# Autodesk Inventor assembly: Shoulder Joint Assembly
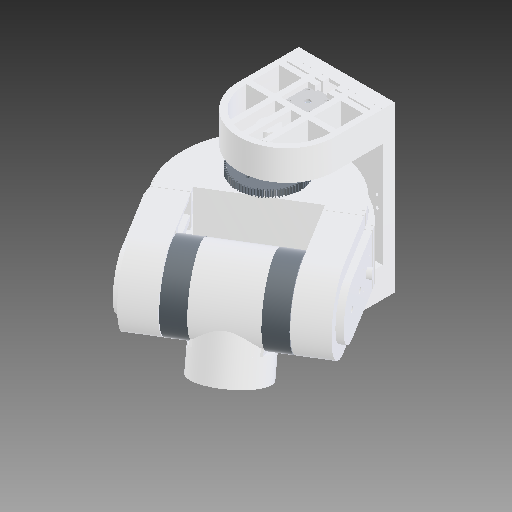
[picture p0: Inventor's stored thumbnail of the model, 512x512]
Saved by Autodesk Inventor 2017 SP1 (Build 210196100, 196)
## iProperties
Created: 2017-06-01
Part Number: Shoulder Joint Assembly
Document SubType Name: Assembly
Designer: Zach
Author: Zach
## Documents named in this file (22)
- C:\Users\Zach\Documents\GitHub\cr-laundry-robot\src\Body\Arm Assembly\Shoulder Joint Assembly\Shoulder Joint Assembly.iam
- C:\Users\Zach\Documents\GitHub\cr-laundry-robot\src\Body\Arm Assembly\Shoulder Joint Assembly\SJ002.ipt
- C:\Users\Zach\Documents\GitHub\cr-laundry-robot\src\Body\Arm Assembly\Shoulder Joint Assembly\SJ003.ipt
- C:\Users\Zach\Documents\GitHub\cr-laundry-robot\src\Body\Arm Assembly\Shoulder Joint Assembly\SJ001.ipt
- C:\Users\Zach\Documents\GitHub\cr-laundry-robot\lib\Stepper Motor - NEMA 17\NEMA17.ipt
- C:\Users\Zach\Documents\GitHub\cr-laundry-robot\src\Body\Arm Assembly\Shoulder Joint Assembly\SJ004.ipt
- C:\Users\Zach\Documents\GitHub\cr-laundry-robot\src\Body\Arm Assembly\Shoulder Joint Assembly\SJ005.ipt
- C:\Users\Zach\Documents\GitHub\cr-laundry-robot\src\Body\Arm Assembly\Shoulder Joint Assembly\SJ006.ipt
- C:\Users\Zach\Documents\GitHub\cr-laundry-robot\lib\U51105\U51105.ipt
- C:\Users\Zach\Documents\GitHub\cr-laundry-robot\lib\QS12MM250\QS12MM250.ipt
- C:\Users\Zach\Documents\GitHub\cr-laundry-robot\lib\6201RS\6201RS.ipt
- C:\Users\Zach\Documents\GitHub\cr-laundry-robot\src\Body\Arm Assembly\Shoulder Joint Assembly\SJ007.ipt
- C:\Users\Zach\Documents\GitHub\cr-laundry-robot\src\Body\Arm Assembly\Shoulder Joint Assembly\SJ008.ipt
- C:\Users\Zach\Documents\GitHub\cr-laundry-robot\src\Body\Arm Assembly\Shoulder Joint Assembly\Shoulder Joint Assembly\Design Accelerator\Spur Gears1.iam
- C:\Users\Zach\Documents\GitHub\cr-laundry-robot\src\Body\Arm Assembly\Shoulder Joint Assembly\SJ009.ipt
- C:\Users\Zach\Documents\GitHub\cr-laundry-robot\lib\Strain Wave Gearbox\StrainWaveGearbox.iam
- C:\Users\Zach\Documents\GitHub\cr-laundry-robot\src\Body\Arm Assembly\Shoulder Joint Assembly\Motor Gear.ipt
- C:\Users\Zach\Documents\GitHub\cr-laundry-robot\src\Body\Arm Assembly\Shoulder Joint Assembly\Motor Coupler.ipt
- C:\Users\Zach\Documents\GitHub\cr-laundry-robot\src\Body\Arm Assembly\Shoulder Joint Assembly\SJ013.ipt
- C:\Users\Zach\Documents\GitHub\cr-laundry-robot\src\Body\Arm Assembly\Shoulder Joint Assembly\SJ014.ipt
- C:\Users\Zach\Documents\GitHub\cr-laundry-robot\src\Body\Arm Assembly\Shoulder Joint Assembly\SJ016.ipt
- C:\Users\Zach\Documents\GitHub\cr-laundry-robot\lib\22x8x8mm Bearing.ipt
## Components (41 placed, 21 different names)
1. SJ001:1 — Mate:47, Mate:173, Mate:176, Mate:223, Mate:227, Mate:228, Mate:229, Mate:230, Mate:231, Mate:232, Mate:234, Mate:235
2. SJ001:2 — Mate:162, Mate:168, Mate:169, Mate:170, Mate:199, Mate:201, Mate:202, Mate:204, Mate:205, Mate:206, Mate:208, Mate:209, Mate:210, Mate:211, Mate:219
3. SJ002:1 — Mate:1, Mate:4, Mate:8, Mate:9, Mate:174, Mate:178
4. SJ002:2 — Mate:18, Mate:19, Mate:20, Mate:172
5. SJ003:1 — Mate:1, Mate:4, Mate:8, Mate:9, Mate:18, Mate:19, Mate:20, Mate:148, Mate:149, Mate:150, Mate:164, Mate:165, Mate:166, Mate:167, Mate:179, Mate:180, Mate:182
6. SJ004:1 — Mate:130, Mate:162, Mate:163, Mate:209, Mate:210, Mate:211, Mate:212, Mate:213, Mate:214
7. SJ004:2 — Mate:47, Mate:54, Mate:55, Mate:56, Mate:216, Mate:217
8. SJ005:1 — Mate:54, Mate:55, Mate:56, Mate:60, Mate:67, Mate:69, Mate:70, Mate:80, Flush:1, Mate:218
9. SJ005:2 — Mate:68, Mate:82, Mate:84, Mate:130, Mate:136, Flush:1, Mate:163, Mate:214, Mate:218
10. SJ006:2 — Mate:67, Mate:68, Mate:69, Mate:70, Mate:78, Mate:79, Mate:83
11. NEMA17:3 — Mate:148, Mate:149, Mate:150, Mate:181
12. U51105:1 — Mate:131, Mate:139, Mate:215
13. U51105:2 — Mate:78, Mate:79
14. QS12MM250:1 — Mate:80, Mate:105, Mate:117, Mate:119, Mate:120, Mate:132, Mate:134, Mate:215
15. 6201RS:1 — Mate:82, Mate:138
16. 6201RS:2 — Mate:83, Mate:84
17. SJ007:1 — Mate:121, Mate:122, Mate:123, Mate:133
18. SJ008:1 — Mate:119, Mate:125, Mate:126, Mate:127, Mate:132
19. SJ008:2 — Mate:97, Mate:98, Mate:99, Mate:105, Mate:112, Mate:117, Mate:120, Mate:121, Mate:122, Mate:123, Mate:124, Mate:131
20. NEMA17:4 — Mate:97, Mate:98, Mate:99, Mate:137
21. SJ007:2 — Mate:125, Mate:126, Mate:127, Mate:133
22. Spur Gears:1 [sub-assembly] — Mate:134, Mate:136, Mate:137, Mate:138, Mate:139
23. SJ009:1 — Mate:212, Mate:213
24. SJ009:2 — Mate:216, Mate:217
25. StrainWaveGearbox:1 [sub-assembly] — Mate:164, Mate:165, Mate:166
26. StrainWaveGearbox:2 [sub-assembly] — Mate:167, Mate:168, Mate:169, Mate:170, Mate:172
27. StrainWaveGearbox:3 [sub-assembly] — Mate:173, Mate:174, Mate:176, Mate:178
28. Motor Gear:1 — Mate:181, Mate:182, Rotation:1
29. Motor Coupler:1 — Mate:179, Mate:180, Rotation:1
30. SJ013:1 — Mate:203, Mate:204, Mate:207
31. SJ014:1 — Mate:202, Mate:219, Mate:220, Mate:221
32. NEMA17:5 — Mate:199, Mate:201, Mate:203, Mate:207, Mate:208
33. SJ016:1 — Mate:205, Mate:206, Mate:222, Flush:2
34. 22x8x8mm Bearing:1 — Mate:222, Flush:2
35. 22x8x8mm Bearing:2 — Mate:220, Mate:221
36. SJ013:2 — Mate:229, Mate:230
37. SJ014:2 — Mate:223, Mate:224, Mate:225, Mate:231
38. SJ016:2 — Mate:226, Flush:3, Mate:227, Mate:228
39. 22x8x8mm Bearing:4 — Mate:226, Flush:3
40. 22x8x8mm Bearing:5 — Mate:224, Mate:225
41. NEMA17:6 — Mate:232, Mate:234, Mate:235
## Relationships (106: Mate 102, Flush 3, RelateRotation 1)
- Mate:1: SJ002:1 ↔ SJ003:1
- Mate:4: SJ002:1 ↔ SJ003:1
- Mate:8: SJ002:1 ↔ SJ003:1
- Mate:9: SJ002:1 ↔ SJ003:1
- Mate:18: SJ002:2 ↔ SJ003:1
- Mate:19: SJ002:2 ↔ SJ003:1
- Mate:20: SJ002:2 ↔ SJ003:1
- Mate:47: SJ001:1 ↔ SJ004:2
- Mate:54: SJ004:2 ↔ SJ005:1
- Mate:55: SJ004:2 ↔ SJ005:1
- Mate:56: SJ004:2 ↔ SJ005:1
- Mate:60: SJ005:1
- Mate:67: SJ005:1 ↔ SJ006:2
- Mate:68: SJ005:2 ↔ SJ006:2
- Mate:69: SJ005:1 ↔ SJ006:2
- Mate:70: SJ005:1 ↔ SJ006:2
- Mate:78: SJ006:2 ↔ U51105:2
- Mate:79: SJ006:2 ↔ U51105:2
- Mate:80: SJ005:1 ↔ QS12MM250:1
- Mate:82: SJ005:2 ↔ 6201RS:1
- Mate:83: SJ006:2 ↔ 6201RS:2
- Mate:84: SJ005:2 ↔ 6201RS:2
- Mate:97: SJ008:2 ↔ NEMA17:4
- Mate:98: SJ008:2 ↔ NEMA17:4
- Mate:99: SJ008:2 ↔ NEMA17:4
- Mate:105: QS12MM250:1 ↔ SJ008:2
- Mate:112: SJ008:2
- Mate:117: QS12MM250:1 ↔ SJ008:2
- Mate:119: QS12MM250:1 ↔ SJ008:1
- Mate:120: QS12MM250:1 ↔ SJ008:2
- Mate:121: SJ007:1 ↔ SJ008:2
- Mate:122: SJ007:1 ↔ SJ008:2
- Mate:123: SJ007:1 ↔ SJ008:2
- Mate:124: SJ008:2
- Mate:125: SJ008:1 ↔ SJ007:2
- Mate:126: SJ008:1 ↔ SJ007:2
- Mate:127: SJ008:1 ↔ SJ007:2
- Mate:130: SJ004:1 ↔ SJ005:2
- Mate:131: U51105:1 ↔ SJ008:2
- Mate:132: QS12MM250:1 ↔ SJ008:1
- Mate:133: SJ007:1 ↔ SJ007:2
- Mate:134: QS12MM250:1 ↔ Spur Gears:1
- Mate:136: SJ005:2 ↔ Spur Gears:1
- Mate:137: NEMA17:4 ↔ Spur Gears:1
- Mate:138: 6201RS:1 ↔ Spur Gears:1
- Mate:139: U51105:1 ↔ Spur Gears:1
- Mate:148: SJ003:1 ↔ NEMA17:3
- Mate:149: SJ003:1 ↔ NEMA17:3
- Mate:150: SJ003:1 ↔ NEMA17:3
- Mate:162: SJ001:2 ↔ SJ004:1
- Flush:1: SJ005:1 ↔ SJ005:2
- Mate:163: SJ004:1 ↔ SJ005:2
- Mate:164: SJ003:1 ↔ StrainWaveGearbox:1
- Mate:165: SJ003:1 ↔ StrainWaveGearbox:1
- Mate:166: SJ003:1 ↔ StrainWaveGearbox:1
- Mate:167: SJ003:1 ↔ StrainWaveGearbox:2
- Mate:168: SJ001:2 ↔ StrainWaveGearbox:2
- Mate:169: SJ001:2 ↔ StrainWaveGearbox:2
- Mate:170: SJ001:2 ↔ StrainWaveGearbox:2
- Mate:172: SJ002:2 ↔ StrainWaveGearbox:2
- Mate:173: SJ001:1 ↔ StrainWaveGearbox:3
- Mate:174: SJ002:1 ↔ StrainWaveGearbox:3
- Mate:176: SJ001:1 ↔ StrainWaveGearbox:3
- Mate:178: SJ002:1 ↔ StrainWaveGearbox:3
- Mate:179: SJ003:1 ↔ Motor Coupler:1
- Mate:180: SJ003:1 ↔ Motor Coupler:1
- Mate:181: NEMA17:3 ↔ Motor Gear:1
- Mate:182: SJ003:1 ↔ Motor Gear:1
- Rotation:1 [RelateRotation] (1 ul): Motor Gear:1 ↔ Motor Coupler:1
- Mate:199: SJ001:2 ↔ NEMA17:5
- Mate:201: SJ001:2 ↔ NEMA17:5
- Mate:202: SJ001:2 ↔ SJ014:1
- Mate:203: SJ013:1 ↔ NEMA17:5
- Mate:204: SJ001:2 ↔ SJ013:1
- Mate:205: SJ001:2 ↔ SJ016:1
- Mate:206: SJ001:2 ↔ SJ016:1
- Mate:207: SJ013:1 ↔ NEMA17:5
- Mate:208: SJ001:2 ↔ NEMA17:5
- Mate:209: SJ001:2 ↔ SJ004:1
- Mate:210: SJ001:2 ↔ SJ004:1
- Mate:211: SJ001:2 ↔ SJ004:1
- Mate:212: SJ004:1 ↔ SJ009:1
- Mate:213: SJ004:1 ↔ SJ009:1
- Mate:214: SJ004:1 ↔ SJ005:2
- Mate:215: U51105:1 ↔ QS12MM250:1
- Mate:216: SJ004:2 ↔ SJ009:2
- Mate:217: SJ004:2 ↔ SJ009:2
- Mate:218: SJ005:1 ↔ SJ005:2
- Mate:219: SJ001:2 ↔ SJ014:1
- Mate:220: SJ014:1 ↔ 22x8x8mm Bearing:2
- Mate:221: SJ014:1 ↔ 22x8x8mm Bearing:2
- Mate:222: SJ016:1 ↔ 22x8x8mm Bearing:1
- Flush:2: SJ016:1 ↔ 22x8x8mm Bearing:1
- Mate:223: SJ001:1 ↔ SJ014:2
- Mate:224: SJ014:2 ↔ 22x8x8mm Bearing:5
- Mate:225: SJ014:2 ↔ 22x8x8mm Bearing:5
- Mate:226: SJ016:2 ↔ 22x8x8mm Bearing:4
- Flush:3: SJ016:2 ↔ 22x8x8mm Bearing:4
- Mate:227: SJ001:1 ↔ SJ016:2
- Mate:228: SJ001:1 ↔ SJ016:2
- Mate:229: SJ001:1 ↔ SJ013:2
- Mate:230: SJ001:1 ↔ SJ013:2
- Mate:231: SJ001:1 ↔ SJ014:2
- Mate:232: SJ001:1 ↔ NEMA17:6
- Mate:234: SJ001:1 ↔ NEMA17:6
- Mate:235: SJ001:1 ↔ NEMA17:6
